# Autodesk Inventor assembly: X-linear bearing shroud
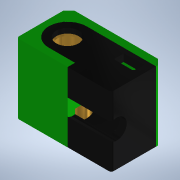
[picture p0: Inventor's stored thumbnail of the model, 180x180]
Saved by Autodesk Inventor 2020.4 (Build 244396000, 396)
## iProperties
Created: 2021-02-25
Part Number: X-linear bearing shroud
Document SubType Name: Assembly
Designer: AOB
Mass: 36.5839 g
Surface Area: 112.043 cm^2
Volume: 13.8686 cm^3
Density: 2.63789 g/cm^3
Author: AOB
## Documents named in this file (4)
- C:\Users\marti\Documents\Inventor\ProjectBoron\Boron Ultima\X-linear bearing shroud.iam
- C:\Users\marti\Documents\Inventor\ProjectBoron\Boron Ultima\lm8uu-graphite.ipt
- C:\Users\marti\Documents\Inventor\ProjectBoron\Boron Ultima\X-linear bearing shroud-A.ipt
- C:\Users\marti\Documents\Inventor\ProjectBoron\Boron Ultima\X-linear bearing shroud-B.ipt
## Components (3 placed, 3 different names)
1. X-linear bearing shroud-B:2 — Rigid:1
2. X-linear bearing shroud-A:1 — Rigid:1, Mate:1, Mate:2
3. lm8uu-graphite:1 — Mate:1, Mate:2
## Relationships (4: Mate 2, Flush 1, WeldJoint 1)
- [Flush]: X-linear bearing shroud-B:2 ↔ X-linear bearing shroud-A:1
- Rigid:1 [WeldJoint]: X-linear bearing shroud-B:2 ↔ X-linear bearing shroud-A:1
- Mate:1: X-linear bearing shroud-A:1 ↔ lm8uu-graphite:1
- Mate:2: X-linear bearing shroud-A:1 ↔ lm8uu-graphite:1
